# Autodesk Inventor assembly: aerospike assembly
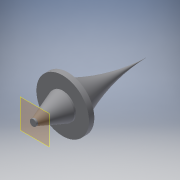
[picture p0: Inventor's stored thumbnail of the model, 180x180]
Saved by Autodesk Inventor 2017 (Build 210142000, 142)
## iProperties
Created: 2016-10-16
Part Number: aerospike assembly
Document SubType Name: Assembly
Designer: Will
Author: Will
## Documents named in this file (3)
- C:\Users\Will\Documents\Inventor\Aerospike\aerospike assembly.iam
- C:\Users\Will\Documents\Inventor\Aerospike\Spike tip.ipt
- C:\Users\Will\Documents\Inventor\Aerospike\Aerospike base.ipt
## Components (2 placed, 2 different names)
1. Spike tip:1 — Insert:1
2. Aerospike base:1 — Insert:1
## Relationships (1: Insert 1)
- Insert:1: Spike tip:1 ↔ Aerospike base:1
